# Autodesk Inventor assembly: BELT_SUPPORT_INNER
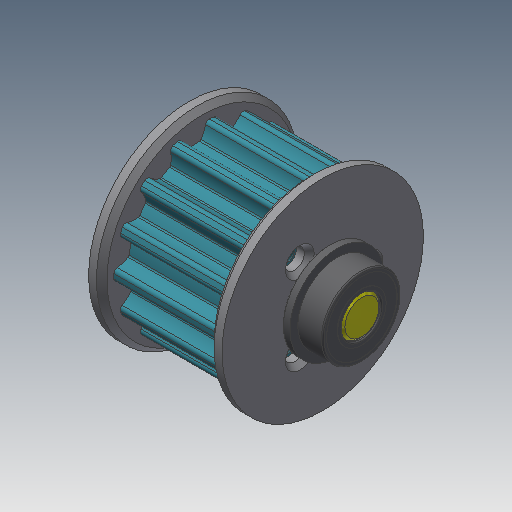
[picture p0: Inventor's stored thumbnail of the model, 512x512]
Saved by Autodesk Inventor 2019.4 (Build 234330000, 330)
## iProperties
Created: 2019-11-12
Part Number: BELT_SUPPORT_INNER
Material: 一般
Document SubType Name: Assembly
Designer: y6tada
Mass: 1.29772 g
Surface Area: 26.4675 cm^2
Volume: 1.29772 cm^3
Density: 1 g/cm^3
Author: y6tada
## Documents named in this file (6)
- C:\Workspace\Yuni9\Inventor\Asm\UPPER_LEG\BELT_SUPPORT_INNER.iam
- C:\Workspace\Yuni9\Inventor\Asm\TIMING_PULLEY\TIMING_BELT_P15.ipt
- C:\Workspace\Yuni9\Inventor\Asm\UPPER_LEG\SHAFT_3x15.ipt
- C:\Workspace\Yuni9\Inventor\Libs\NSK Bearing\NSK_RB_MF63ZZ\MF63ZZ.iam
- C:\Workspace\Yuni9\Inventor\Asm\UPPER_LEG\INNER_TIMING_PULLEY_COVER.ipt
- C:\Workspace\Yuni9\Inventor\Asm\UPPER_LEG\CB-301.5PC.ipt
## Components (8 placed, 5 different names)
1. TIMING_BELT_P15:1 — メイト:1, フラッシュ:1, フラッシュ:2, メイト:2, フラッシュ:4, メイト:13, メイト:15
2. SHAFT_3x15:1 — フラッシュ:3, メイト:2, メイト:3, メイト:7, メイト:14, メイト:16, メイト:17
3. MF63ZZ:1 [sub-assembly] — メイト:3, メイト:9
4. INNER_TIMING_PULLEY_COVER:1 — メイト:5, メイト:6, フラッシュ:4, メイト:8
5. CB-301.5PC:1 — メイト:7, メイト:8, メイト:9
6. MF63ZZ:2 [sub-assembly] — メイト:11, メイト:16
7. INNER_TIMING_PULLEY_COVER:2 — メイト:12, メイト:13, メイト:14, メイト:15
8. CB-301.5PC:2 — メイト:11, メイト:12, メイト:17
## Relationships (19: Mate 15, Flush 4)
- メイト:1 [Mate]: TIMING_BELT_P15:1
- フラッシュ:1 [Flush]: TIMING_BELT_P15:1
- フラッシュ:2 [Flush]: TIMING_BELT_P15:1
- フラッシュ:3 [Flush]: SHAFT_3x15:1
- メイト:2 [Mate]: TIMING_BELT_P15:1 ↔ SHAFT_3x15:1
- メイト:3 [Mate]: SHAFT_3x15:1 ↔ MF63ZZ:1
- メイト:5 [Mate]: INNER_TIMING_PULLEY_COVER:1
- メイト:6 [Mate]: INNER_TIMING_PULLEY_COVER:1
- フラッシュ:4 [Flush]: TIMING_BELT_P15:1 ↔ INNER_TIMING_PULLEY_COVER:1
- メイト:7 [Mate]: SHAFT_3x15:1 ↔ CB-301.5PC:1
- メイト:8 [Mate]: INNER_TIMING_PULLEY_COVER:1 ↔ CB-301.5PC:1
- メイト:9 [Mate]: MF63ZZ:1 ↔ CB-301.5PC:1
- メイト:11 [Mate]: MF63ZZ:2 ↔ CB-301.5PC:2
- メイト:12 [Mate]: INNER_TIMING_PULLEY_COVER:2 ↔ CB-301.5PC:2
- メイト:13 [Mate]: TIMING_BELT_P15:1 ↔ INNER_TIMING_PULLEY_COVER:2
- メイト:14 [Mate]: SHAFT_3x15:1 ↔ INNER_TIMING_PULLEY_COVER:2
- メイト:15 [Mate]: TIMING_BELT_P15:1 ↔ INNER_TIMING_PULLEY_COVER:2
- メイト:16 [Mate]: SHAFT_3x15:1 ↔ MF63ZZ:2
- メイト:17 [Mate]: SHAFT_3x15:1 ↔ CB-301.5PC:2
